# Autodesk Inventor assembly: Drive Assembly
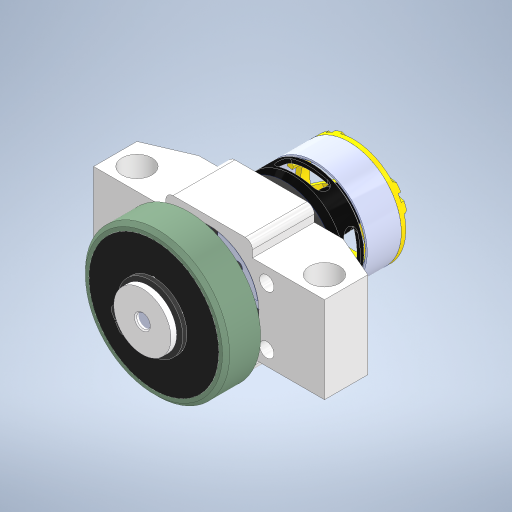
[picture p0: Inventor's stored thumbnail of the model, 512x512]
Saved by Autodesk Inventor 2023.2 (Build 272271000, 271)
## iProperties
Created: 2023-04-12
Part Number: Drive Assembly
Document SubType Name: Assembly
Designer: Nathan Cai
Mass: 34.861 g
Surface Area: 143.766 cm^2
Volume: 13.0781 cm^3
Density: 2.66561 g/cm^3
Author: Nathan Cai
## Documents named in this file (4)
- C:\Users\Nathan Cai\Documents\Inventor\Flatbread V1.0\Drive Assembly.iam
- C:\Users\Nathan Cai\Documents\Inventor\Flatbread V1.0\Custom Wheel V2.0\Recessed Wheels V2.0.iam
- C:\Users\Nathan Cai\Documents\Inventor\Flatbread V1.0\Motor Sleeve.ipt
- C:\Users\Nathan Cai\Documents\Inventor\Flatbread V1.0\RR Brushless\RR-Brushless-Planetary.iam
## Components (3 placed, 3 different names)
1. Recessed Wheels V2.0:1 [sub-assembly]
2. Motor Sleeve:1 — Mate:1, Flush:1
3. RR-Brushless-Planetary:1 [sub-assembly] — Mate:1, Flush:1
## Relationships (2: Mate 1, Flush 1)
- Mate:1: Motor Sleeve:1 ↔ RR-Brushless-Planetary:1
- Flush:1: Motor Sleeve:1 ↔ RR-Brushless-Planetary:1
